# Autodesk Inventor assembly: bike-rack-assembly
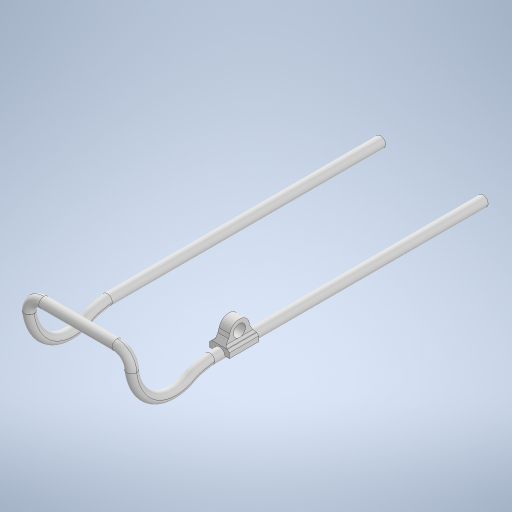
[picture p0: Inventor's stored thumbnail of the model, 512x512]
Saved by Autodesk Inventor 2024.1 (Build 281209000, 209)
## iProperties
Created: 2025-08-15
Part Number: bike-rack-assembly
Document SubType Name: Assembly
Designer: iwheard
Author: iwheard
## Documents named in this file (3)
- C:\Users\iwheard\Documents\0004-CAD\3D-cad-main\bike-rack\bike-rack-assembly.iam
- C:\Users\iwheard\Documents\0004-CAD\3D-cad-main\bike-rack\bike-rack.ipt
- C:\Users\iwheard\Documents\0004-CAD\3D-cad-main\h6-case\rack-mounts.ipt
## Components (2 placed, 2 different names)
1. bike-rack:1 — Flush:1, Mate:1, Flush:2
2. rack-mounts:1 — Flush:1, Mate:1, Flush:2
## Relationships (3: Flush 2, Mate 1)
- Flush:1: bike-rack:1 ↔ rack-mounts:1
- Mate:1: bike-rack:1 ↔ rack-mounts:1
- Flush:2 (-240 mm): bike-rack:1 ↔ rack-mounts:1
